# Autodesk Inventor assembly: Remote Assembly
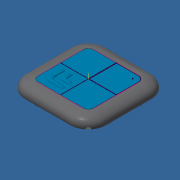
[picture p0: Inventor's stored thumbnail of the model, 180x180]
Saved by Autodesk Inventor 2016 (Build 200138000, 138)
## iProperties
Created: 2015-06-16
Part Number: Remote Assembly
Document SubType Name: Assembly
Designer: Samuel Clay
Author: Samuel Clay
## Documents named in this file (7)
- Z:\remote\enclosure\inventor\Remote Assembly.iam
- Z:\remote\enclosure\inventor\Remote Top.ipt
- Z:\remote\enclosure\inventor\Remote Bottom.ipt
- Z:\remote\enclosure\inventor\Remote Buttons.ipt
- Z:\remote\enclosure\inventor\Eagle PCB rev 21.ipt
- Z:\remote\enclosure\inventor\Case Bottom.ipt
- Z:\remote\enclosure\inventor\Case Top.ipt
## Components (6 placed, 6 different names)
1. Case Top:1
2. Remote Top:1 — Flush:1, Mate:1
3. Remote Buttons:1 — Flush:1, Mate:1
4. Eagle PCB rev 21:1
5. Remote Bottom:1
6. Case Bottom:1
## Relationships (2: Flush 1, Mate 1)
- Flush:1: Remote Top:1 ↔ Remote Buttons:1
- Mate:1: Remote Top:1 ↔ Remote Buttons:1
